# Autodesk Inventor assembly: BasePulleyAssembly
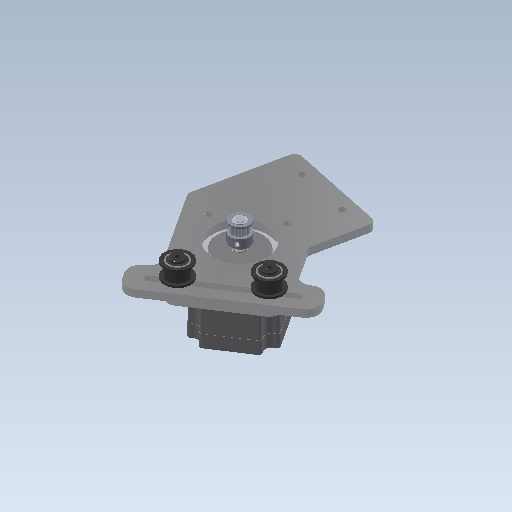
[picture p0: Inventor's stored thumbnail of the model, 512x512]
Saved by Autodesk Inventor 2020.4 (Build 244396010, 396A)
## iProperties
Created: 2021-09-27
Part Number: BasePulleyAssembly
Document SubType Name: Assembly
Designer: justi
Author: justi
## Documents named in this file (6)
- D:\UQ Engineering\2021 ~ 5th Year\Semester 2\METR4911-THESIS\FarmBot CAD\FarmBotV1\BasePulleyAssembly.iam
- D:\UQ Engineering\2021 ~ 5th Year\Semester 2\METR4911-THESIS\FarmBot CAD\FarmBotV1\NEMA 23 - 56mm.iam
- D:\UQ Engineering\2021 ~ 5th Year\Semester 2\METR4911-THESIS\FarmBot CAD\FarmBotV1\GT2 Timing Pulley, Configurable, 20T W6 B5.iam
- D:\UQ Engineering\2021 ~ 5th Year\Semester 2\METR4911-THESIS\FarmBot CAD\FarmBotV1\VSlotHardware\Idler pulley kit.iam
- D:\UQ Engineering\2021 ~ 5th Year\Semester 2\METR4911-THESIS\FarmBot CAD\FarmBotV1\NEMA23MountPlatev5.ipt
- D:\UQ Engineering\2021 ~ 5th Year\Semester 2\METR4911-THESIS\FarmBot CAD\FarmBotV1\BaseTensionBracket.ipt
## Components (6 placed, 5 different names)
1. NEMA 23 - 56mm:1 [sub-assembly] — Mate:5, Mate:6, Mate:7, Mate:8, Mate:14
2. GT2 Timing Pulley, Configurable, 20T W6 B5:1 [sub-assembly] — Mate:5, Flush:2
3. Idler pulley kit:2 [sub-assembly] — Flush:2, Flush:3, Mate:9, Mate:12
4. Idler pulley kit:3 [sub-assembly] — Flush:3, Mate:10, Flush:4, Mate:11
5. NEMA23MountPlatev5:1 — Mate:6, Mate:7, Mate:8, Mate:9, Mate:10, Flush:4, Mate:13
6. BaseTensionBracket:1 — Mate:11, Mate:12, Mate:13, Mate:14
## Relationships (13: Mate 10, Flush 3)
- Mate:5: NEMA 23 - 56mm:1 ↔ GT2 Timing Pulley, Configurable, 20T W6 B5:1
- Flush:2: GT2 Timing Pulley, Configurable, 20T W6 B5:1 ↔ Idler pulley kit:2
- Flush:3: Idler pulley kit:2 ↔ Idler pulley kit:3
- Mate:6: NEMA 23 - 56mm:1 ↔ NEMA23MountPlatev5:1
- Mate:7: NEMA 23 - 56mm:1 ↔ NEMA23MountPlatev5:1
- Mate:8: NEMA 23 - 56mm:1 ↔ NEMA23MountPlatev5:1
- Mate:9: Idler pulley kit:2 ↔ NEMA23MountPlatev5:1
- Mate:10: Idler pulley kit:3 ↔ NEMA23MountPlatev5:1
- Flush:4 (-3 mm): Idler pulley kit:3 ↔ NEMA23MountPlatev5:1
- Mate:11: Idler pulley kit:3 ↔ BaseTensionBracket:1
- Mate:12: Idler pulley kit:2 ↔ BaseTensionBracket:1
- Mate:13: NEMA23MountPlatev5:1 ↔ BaseTensionBracket:1
- Mate:14: NEMA 23 - 56mm:1 ↔ BaseTensionBracket:1
